# Autodesk Inventor assembly: Instrument
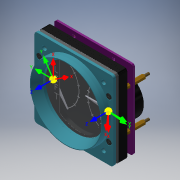
[picture p0: Inventor's stored thumbnail of the model, 180x180]
Saved by Autodesk Inventor 2019 (Build 230136000, 136)
## iProperties
Created: 2018-04-27
Part Number: Instrument
Document SubType Name: Assembly
Designer: Fierl
Author: Fierl
## Documents named in this file (15)
- C:\Users\Fierl\OneDrive - Van Ierland\Documents\Inventor\FlightSim\Instrument.iam
- C:\Users\Fierl\OneDrive - Van Ierland\Documents\Inventor\FlightSim\Front Ring.ipt
- C:\Users\Fierl\OneDrive - Van Ierland\Documents\Inventor\FlightSim\FrontGlass.ipt
- C:\Users\Fierl\OneDrive - Van Ierland\Documents\Inventor\FlightSim\FrontMask.ipt
- C:\Users\Fierl\OneDrive - Van Ierland\Documents\Inventor\FlightSim\Spacer-M2.ipt
- C:\Users\Fierl\OneDrive - Van Ierland\Documents\Inventor\FlightSim\stepper_pcb.iam
- C:\Users\Fierl\OneDrive - Van Ierland\Documents\Inventor\FlightSim\filler_ring.ipt
- C:\Users\Fierl\OneDrive - Van Ierland\Documents\Inventor\FlightSim\dail_face.ipt
- C:\Users\Fierl\OneDrive - Van Ierland\Documents\Inventor\FlightSim\Spacer\Spacer-M2-05.ipt
- C:\Users\Fierl\Documents\Inventor\Content Center Files\R2019\en-US\ISO 7046-2 H\ISO 7046-2 H - M2x14 - 8.8 - H1.ipt
- C:\Users\Fierl\Documents\Inventor\Content Center Files\R2019\en-US\AS 1474(1)\AS 1474 - M2(1).ipt
- C:\Users\Fierl\OneDrive - Van Ierland\Documents\Inventor\FlightSim\SpacerRing\filler_ring-03.ipt
- C:\Users\Fierl\OneDrive - Van Ierland\Documents\Inventor\FlightSim\SpacerRing\filler_ring-02.ipt
- C:\Users\Fierl\OneDrive - Van Ierland\Documents\Inventor\FlightSim\Spacer\Spacer-M2-10.ipt
- C:\Users\Fierl\OneDrive - Van Ierland\Documents\Inventor\FlightSim\Instrument.xlsx
## Components (20 placed, 11 different names)
1. Front Ring:1 — Mate:1, Flush:1, Flush:2, Flush:6, Flush:16, Flush:17, Flush:18, Mate:6, Flush:19, Flush:20, Mate:7, Flush:21, Flush:22, Flush:23, Flush:24, Flush:25, Flush:26
2. FrontGlass:1 — Mate:1, Flush:1, Flush:2, Flush:3, Flush:4, Flush:7, Flush:9, Flush:10, Flush:11, Mate:6, Flush:19, Flush:20
3. FrontMask:2 — Flush:3, Flush:4, Mate:8
4. stepper_pcb:1 [sub-assembly] — Flush:7, Flush:9, Insert:3, Insert:4, Insert:5, Insert:6
5. filler_ring-02:3 — Flush:10, Flush:11, Mate:10, Flush:22, Flush:23
6. DailFace:1 — Mate:9, Mate:10, Flush:25, Flush:26
7. Spacer-M2-05:2 — Insert:3, Insert:14
8. Spacer-M2-05:3 — Insert:4, Insert:8, Insert:12
9. Spacer-M2-05:4 — Insert:5, Insert:15
10. Spacer-M2-05:5 — Insert:6, Insert:13
11. filler_ring-03:2 — Mate:8, Mate:9, Flush:21, Flush:24
12. AS 1474 - Metric M2:1
13. Spacer-M2-10:6 — Insert:12
14. Spacer-M2-10:7 — Insert:13
15. Spacer-M2-10:8 — Insert:14
16. Spacer-M2-10:9 — Insert:15
17. ISO 7046-2 H M2x14 - 8.8 - H1:1 — Flush:6, Insert:8, Mate:7
18. ISO 7046-2 H M2x14 - 8.8 - H1:2
19. ISO 7046-2 H M2x14 - 8.8 - H1:3
20. ISO 7046-2 H M2x14 - 8.8 - H1:4
## Component patterns: (4 elements, first: ISO 7046-2 H M2x14 - 8.8 - H1:1)
## Relationships (35: Flush 20, Insert 9, Mate 6)
- Mate:1: Front Ring:1 ↔ FrontGlass:1
- Flush:1: Front Ring:1 ↔ FrontGlass:1
- Flush:2: Front Ring:1 ↔ FrontGlass:1
- Flush:3: FrontGlass:1 ↔ FrontMask:2
- Flush:4: FrontGlass:1 ↔ FrontMask:2
- Flush:6: Front Ring:1 ↔ ISO 7046-2 H M2x14 - 8.8 - H1:1
- Flush:7: FrontGlass:1 ↔ stepper_pcb:1
- Flush:9: FrontGlass:1 ↔ stepper_pcb:1
- Flush:10: FrontGlass:1 ↔ filler_ring-02:3
- Flush:11: FrontGlass:1 ↔ filler_ring-02:3
- Insert:3: stepper_pcb:1 ↔ Spacer-M2-05:2
- Insert:4: stepper_pcb:1 ↔ Spacer-M2-05:3
- Insert:5: stepper_pcb:1 ↔ Spacer-M2-05:4
- Insert:6: stepper_pcb:1 ↔ Spacer-M2-05:5
- Insert:8: Spacer-M2-05:3 ↔ ISO 7046-2 H M2x14 - 8.8 - H1:1
- Flush:16: Front Ring:1
- Flush:17: Front Ring:1
- Flush:18: Front Ring:1
- Mate:6: Front Ring:1 ↔ FrontGlass:1
- Flush:19: Front Ring:1 ↔ FrontGlass:1
- Flush:20: Front Ring:1 ↔ FrontGlass:1
- Mate:7: Front Ring:1 ↔ ISO 7046-2 H M2x14 - 8.8 - H1:1
- Insert:12 (-2.5 mm): Spacer-M2-05:3 ↔ Spacer-M2-10:6
- Insert:13 (-2.5 mm): Spacer-M2-05:5 ↔ Spacer-M2-10:7
- Insert:14 (-2.5 mm): Spacer-M2-05:2 ↔ Spacer-M2-10:8
- Insert:15 (-2.5 mm): Spacer-M2-05:4 ↔ Spacer-M2-10:9
- Mate:8: FrontMask:2 ↔ filler_ring-03:2
- Mate:9: DailFace:1 ↔ filler_ring-03:2
- Mate:10: filler_ring-02:3 ↔ DailFace:1
- Flush:21: Front Ring:1 ↔ filler_ring-03:2
- Flush:22: Front Ring:1 ↔ filler_ring-02:3
- Flush:23: Front Ring:1 ↔ filler_ring-02:3
- Flush:24: Front Ring:1 ↔ filler_ring-03:2
- Flush:25: Front Ring:1 ↔ DailFace:1
- Flush:26: Front Ring:1 ↔ DailFace:1
## Named parameters: circle_dimension = 56 mm, circle_dimension_inner = 47 mm, hole_from_center = 63.5 mm, hole_distance = 22.45064 mm, backplate_width = 60 mm, ring_depth = 6 mm, ring_thickness = 9 mm, ring_top_thickness = 2 mm, ring_outer_bevel_height = 3 mm, ring_outer_bevel_depth = 0.5 mm, ring_inner_bevel_depth = 3.5 mm, screw_distance_center = 15 mm, screw_distance_outside = 3.5 mm, front_plate_thickness = 2 mm, glass_thickness = 2 mm, encoders = 0, encoder_axis = 8 mm, encoder_emboss = 0, encoder_width = 27 mm, encoder_rad = 49 mm, encoder_extrude_hight = 3 mm, mask_width = 30 mm, pointer_length = 18 mm, pointer_axis = 1 mm, pointer_axis_outside = 3 mm
